# Autodesk Inventor assembly: FInished_Assembly_Mk
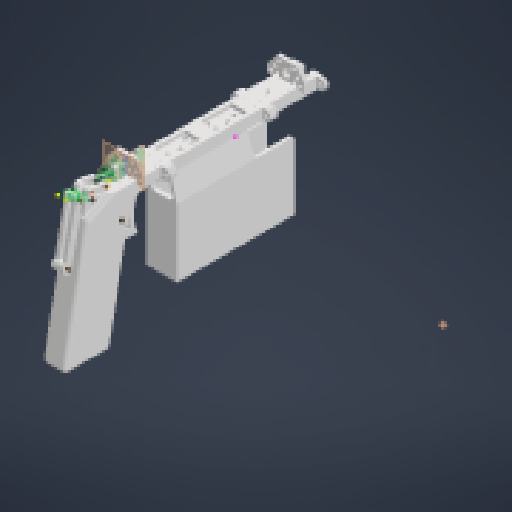
[picture p0: Inventor's stored thumbnail of the model, 512x512]
Saved by Autodesk Inventor 2024.1 (Build 281209000, 209)
## iProperties
Created: 2023-08-18
Part Number: FInished_Assembly_Mk
Document SubType Name: Assembly
Designer: Eleanor
Author: Eleanor
## Documents named in this file (11)
- C:\Users\Eleanor\Documents\Inventor\4.5mm ERS\FInished_Assembly_Mk.iam
- C:\Users\Eleanor\Documents\Inventor\4.5mm ERS\DoubleLengthCarrier.iam
- C:\Users\Eleanor\Documents\Inventor\4.5mm ERS\SlottedCarrierFull.ipt
- C:\Users\Eleanor\Documents\Inventor\4.5mm ERS\CapacitorBank.ipt.iam
- C:\Users\Eleanor\Documents\Inventor\4.5mm ERS\WireBarrelComponent.iam
- C:\Users\Eleanor\Documents\Inventor\4.5mm ERS\TestAssembly_02.iam
- GripAssembly MK.001.iam
- C:\Users\Eleanor\Documents\Inventor\Content Center Files\R2024\en-US\ISO 7380-1\ISO 7380-1 - M3 x 8.ipt
- C:\Users\Eleanor\Documents\Inventor\Content Center Files\R2024\en-US\ISO 7380-1\ISO 7380-1 - M3 x 10.ipt
- C:\Users\Eleanor\Documents\Inventor\Content Center Files\R2024\en-US\ISO 7380-1\ISO 7380-1 - M3 x 12.ipt
- CapacitorBank.ipt
## Components (20 placed, 8 different names)
1. DoubleLengthCarrier:1 [sub-assembly] — Mate:7, Mate:8, Mate:12, Mate:27, Mate:28, Mate:29, Mate:30, Mate:31, Mate:32, Mate:39, Mate:54, Mate:72, Mate:79, Mate:80, Mate:94, Mate:95, Mate:96, Mate:97, Mate:102, Mate:103, Mate:104, Mate:105
2. SlottedCarrierFull:1 — Mate:5, Mate:6, Mate:7, Mate:8, Mate:9, Mate:11, Mate:12, Mate:13, Mate:14, Mate:15, Mate:68, Mate:70, Mate:92, Mate:93, Mate:98, Mate:99
3. CapacitorBank.ipt:1 [sub-assembly] — Mate:27, Mate:28
4. WireBarrelComponent:1 [sub-assembly] — Mate:5, Mate:6, Mate:11, Mate:13, Mate:14, Mate:15, Mate:56, Mate:58, Mate:60, Mate:62, Mate:64, Mate:66, Mate:76, Mate:77, Mate:100, Mate:101
5. GripAssembly MK.001:1 [sub-assembly] — Mate:29, Mate:30, Mate:31, Mate:33, Mate:34, Mate:35, Mate:36, Mate:37, Mate:38, Mate:40, Mate:42, Mate:44, Mate:46, Mate:48, Mate:50, Mate:52, Mate:74, Mate:82, Mate:83, Mate:84, Mate:85, Mate:86, Mate:87, Mate:88, Mate:89, Mate:90, Mate:91
6. ISO 7380-1 M3 x 10:1
7. ISO 7380-1 M3 x 12:1 — Mate:102, Mate:103
8. ISO 7380-1 M3 x 8:2
9. ISO 7380-1 M3 x 8:3 — Mate:82, Mate:83
10. ISO 7380-1 M3 x 8:4 — Mate:84, Mate:85
11. ISO 7380-1 M3 x 8:5 — Mate:86, Mate:87
12. ISO 7380-1 M3 x 8:6 — Mate:90
13. ISO 7380-1 M3 x 8:7 — Mate:91
14. ISO 7380-1 M3 x 8:8 — Mate:88, Mate:89
15. ISO 7380-1 M3 x 10:2 — Mate:95, Mate:96
16. ISO 7380-1 M3 x 10:3 — Mate:94, Mate:97
17. ISO 7380-1 M3 x 10:4 — Mate:93, Mate:99
18. ISO 7380-1 M3 x 10:5 — Mate:92, Mate:98
19. ISO 7380-1 M3 x 10:6 — Mate:100, Mate:101
20. ISO 7380-1 M3 x 12:2 — Mate:104, Mate:105
## Relationships (89: Mate 89)
- Mate:5: SlottedCarrierFull:1 ↔ WireBarrelComponent:1
- Mate:6: SlottedCarrierFull:1 ↔ WireBarrelComponent:1
- Mate:7: DoubleLengthCarrier:1 ↔ SlottedCarrierFull:1
- Mate:8: DoubleLengthCarrier:1 ↔ SlottedCarrierFull:1
- Mate:9: SlottedCarrierFull:1
- Mate:11: SlottedCarrierFull:1 ↔ WireBarrelComponent:1
- Mate:12: DoubleLengthCarrier:1 ↔ SlottedCarrierFull:1
- Mate:13: SlottedCarrierFull:1 ↔ WireBarrelComponent:1
- Mate:14: SlottedCarrierFull:1 ↔ WireBarrelComponent:1
- Mate:15: SlottedCarrierFull:1 ↔ WireBarrelComponent:1
- Mate:27: DoubleLengthCarrier:1 ↔ CapacitorBank.ipt:1
- Mate:28: DoubleLengthCarrier:1 ↔ CapacitorBank.ipt:1
- Mate:29: DoubleLengthCarrier:1 ↔ GripAssembly MK.001:1
- Mate:30: DoubleLengthCarrier:1 ↔ GripAssembly MK.001:1
- Mate:31: DoubleLengthCarrier:1 ↔ GripAssembly MK.001:1
- Mate:32: DoubleLengthCarrier:1
- Mate:33: GripAssembly MK.001:1
- Mate:34: GripAssembly MK.001:1
- Mate:35: GripAssembly MK.001:1
- Mate:36: GripAssembly MK.001:1
- Mate:37: GripAssembly MK.001:1
- Mate:38: GripAssembly MK.001:1
- Mate:39: DoubleLengthCarrier:1
- Mate:40: GripAssembly MK.001:1
- Mate:41
- Mate:42: GripAssembly MK.001:1
- Mate:43
- Mate:44: GripAssembly MK.001:1
- Mate:45
- Mate:46: GripAssembly MK.001:1
- Mate:47
- Mate:48: GripAssembly MK.001:1
- Mate:49
- Mate:50: GripAssembly MK.001:1
- Mate:51
- Mate:52: GripAssembly MK.001:1
- Mate:53
- Mate:54: DoubleLengthCarrier:1
- Mate:55
- Mate:56: WireBarrelComponent:1
- Mate:57
- Mate:58: WireBarrelComponent:1
- Mate:59
- Mate:60: WireBarrelComponent:1
- Mate:61
- Mate:62: WireBarrelComponent:1
- Mate:63
- Mate:64: WireBarrelComponent:1
- Mate:65
- Mate:66: WireBarrelComponent:1
- Mate:67
- Mate:68: SlottedCarrierFull:1
- Mate:69
- Mate:70: SlottedCarrierFull:1
- Mate:71
- Mate:72: DoubleLengthCarrier:1
- Mate:73
- Mate:74: GripAssembly MK.001:1
- Mate:75
- Mate:76: WireBarrelComponent:1
- Mate:77: WireBarrelComponent:1
- Mate:78
- Mate:79: DoubleLengthCarrier:1
- Mate:80: DoubleLengthCarrier:1
- Mate:81
- Mate:82: GripAssembly MK.001:1 ↔ ISO 7380-1 M3 x 8:3
- Mate:83: GripAssembly MK.001:1 ↔ ISO 7380-1 M3 x 8:3
- Mate:84: GripAssembly MK.001:1 ↔ ISO 7380-1 M3 x 8:4
- Mate:85: GripAssembly MK.001:1 ↔ ISO 7380-1 M3 x 8:4
- Mate:86: GripAssembly MK.001:1 ↔ ISO 7380-1 M3 x 8:5
- Mate:87: GripAssembly MK.001:1 ↔ ISO 7380-1 M3 x 8:5
- Mate:88: GripAssembly MK.001:1 ↔ ISO 7380-1 M3 x 8:8
- Mate:89: GripAssembly MK.001:1 ↔ ISO 7380-1 M3 x 8:8
- Mate:90: GripAssembly MK.001:1 ↔ ISO 7380-1 M3 x 8:6
- Mate:91: GripAssembly MK.001:1 ↔ ISO 7380-1 M3 x 8:7
- Mate:92: SlottedCarrierFull:1 ↔ ISO 7380-1 M3 x 10:5
- Mate:93: SlottedCarrierFull:1 ↔ ISO 7380-1 M3 x 10:4
- Mate:94: DoubleLengthCarrier:1 ↔ ISO 7380-1 M3 x 10:3
- Mate:95: DoubleLengthCarrier:1 ↔ ISO 7380-1 M3 x 10:2
- Mate:96: DoubleLengthCarrier:1 ↔ ISO 7380-1 M3 x 10:2
- Mate:97: DoubleLengthCarrier:1 ↔ ISO 7380-1 M3 x 10:3
- Mate:98: SlottedCarrierFull:1 ↔ ISO 7380-1 M3 x 10:5
- Mate:99: SlottedCarrierFull:1 ↔ ISO 7380-1 M3 x 10:4
- Mate:100: WireBarrelComponent:1 ↔ ISO 7380-1 M3 x 10:6
- Mate:101: WireBarrelComponent:1 ↔ ISO 7380-1 M3 x 10:6
- Mate:102: DoubleLengthCarrier:1 ↔ ISO 7380-1 M3 x 12:1
- Mate:103: DoubleLengthCarrier:1 ↔ ISO 7380-1 M3 x 12:1
- Mate:104: DoubleLengthCarrier:1 ↔ ISO 7380-1 M3 x 12:2
- Mate:105: DoubleLengthCarrier:1 ↔ ISO 7380-1 M3 x 12:2
